# Autodesk Inventor assembly: TheHat
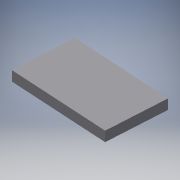
[picture p0: Inventor's stored thumbnail of the model, 180x180]
Saved by Autodesk Inventor 2017 (Build 210142000, 142)
## iProperties
Created: 2016-09-01
Part Number: TheHat
Document SubType Name: Assembly
Designer: smart
Author: smart
## Documents named in this file (3)
- C:\Users\smart\Documents\GitHub\ClipFanHat\TheHat.iam
- C:\Users\smart\Documents\GitHub\ClipFanHat\Impeller.ipt
- C:\Users\smart\Documents\GitHub\ClipFanHat\main_chassis.ipt
## Components (2 placed, 2 different names)
1. Impeller:1 — Insert:1
2. main_chassis:1 — Insert:1
## Relationships (1: Insert 1)
- Insert:1: Impeller:1 ↔ main_chassis:1
